# Autodesk Inventor assembly: Gantry Assembly
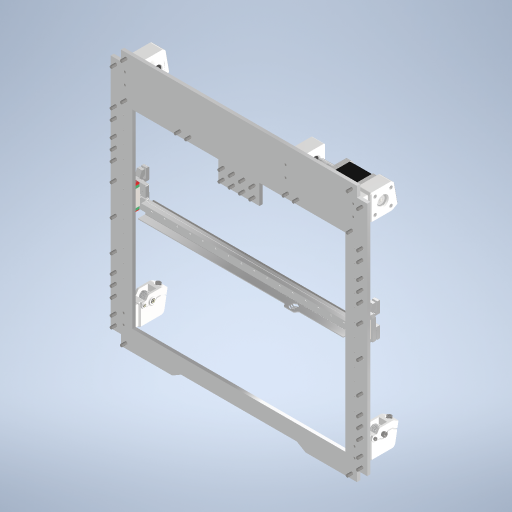
[picture p0: Inventor's stored thumbnail of the model, 512x512]
Saved by Autodesk Inventor 2024 (Build 280153000, 153)
## iProperties
Created: 2024-08-04
Part Number: Gantry Assembly
Document SubType Name: Assembly
Designer: Ishaan
Author: Ishaan
## Documents named in this file (27)
- E:\Projects\Axiom--IDEX-3D-Printer\CAD\04 - Gantry and Y-axis\Gantry Assembly.iam
- E:\Projects\Axiom--IDEX-3D-Printer\CAD\04 - Gantry and Y-axis\Printer Gantry Plate RevI.ipt
- E:\Projects\Axiom--IDEX-3D-Printer\CAD\00 - COTS Components\MGNR12 300mm Rail\MGNR12R100HM\MGNR12R100HM.ipt
- E:\Projects\Axiom--IDEX-3D-Printer\CAD\00 - COTS Components\MGN12H\MGN12H, LINEAR GUIDE BLOCK.ipt
- E:\Projects\Axiom--IDEX-3D-Printer\CAD\00 - COTS Components\MGNR12 400mm Rail\MGNR12R400HM.ipt
- E:\Projects\Axiom--IDEX-3D-Printer\CAD\04 - Gantry and Y-axis\Y-axis Motor Block.ipt
- E:\Projects\Axiom--IDEX-3D-Printer\CAD\00 - COTS Components\NEMA 17 - Y-Axis\NEMA 17 Y-axis.ipt
- E:\Projects\Axiom--IDEX-3D-Printer\CAD\00 - COTS Components\9mm 20T GT2 Timing Pulley 5mm Bore\9mm 20T GT2 Timing Pulley 5mm Bore.ipt
- E:\Projects\Axiom--IDEX-3D-Printer\CAD\04 - Gantry and Y-axis\Y-axis Bearing Pulley Block.ipt
- E:\Projects\Axiom--IDEX-3D-Printer\CAD\00 - COTS Components\608-2RS\608-2RS Bearing.ipt
- E:\Projects\Axiom--IDEX-3D-Printer\CAD\00 - COTS Components\9mm 20T GT2 Timing Pulley 8mm Bore\9mm 20T GT2 Timing Pulley 8mm Bore.ipt
- E:\Projects\Axiom--IDEX-3D-Printer\CAD\04 - Gantry and Y-axis\Y-axis Shaft Support.ipt
- E:\Projects\Axiom--IDEX-3D-Printer\CAD\00 - COTS Components\5x8 Shaft Coupler\Flexible Coupling 5mm x 8mm.ipt
- E:\Projects\Axiom--IDEX-3D-Printer\CAD\04 - Gantry and Y-axis\Y-axis Power Transfer Shaft 360mm.ipt
- E:\Projects\Axiom--IDEX-3D-Printer\CAD\04 - Gantry and Y-axis\R2 Idler Block Left.ipt
- E:\Projects\Axiom--IDEX-3D-Printer\CAD\04 - Gantry and Y-axis\R2 Idler Block Right.ipt
- E:\Projects\Axiom--IDEX-3D-Printer\CAD\00 - COTS Components\9mm 20T GT2 Idler Pulley 5mm Bore\9mm 20T GT2 Idler Pulley 5mm Bore.ipt
- E:\Projects\Axiom--IDEX-3D-Printer\CAD\04 - Gantry and Y-axis\R2 Gantry Bar.ipt
- E:\Projects\Axiom--IDEX-3D-Printer\CAD\04 - Gantry and Y-axis\Gantry Belt Clamp.ipt
- E:\Projects\Axiom--IDEX-3D-Printer\CAD\04 - Gantry and Y-axis\Gantry Stiffener.ipt
- E:\Projects\Axiom--IDEX-3D-Printer\CAD\00 - COTS Components\Hardware\Low Profile M5x16.ipt
- E:\Projects\Axiom--IDEX-3D-Printer\CAD\00 - COTS Components\Hardware\SHCSM5x16.ipt
- E:\Projects\Axiom--IDEX-3D-Printer\CAD\00 - COTS Components\Hardware\SHCSM3x8.ipt
- E:\Projects\Axiom--IDEX-3D-Printer\CAD\00 - COTS Components\Hardware\SHCSM3x25.ipt
- E:\Projects\Axiom--IDEX-3D-Printer\CAD\00 - COTS Components\Hardware\SHCSM5x25.ipt
- E:\Projects\Axiom--IDEX-3D-Printer\CAD\00 - COTS Components\Hardware\M5 LOCKNUT.ipt
- E:\Projects\Axiom--IDEX-3D-Printer\CAD\00 - COTS Components\Hardware\M3 LOCKNUT.ipt
## Components (121 placed, 26 different names)
1. Printer Gantry Plate RevI:1 — Insert:1, Insert:2, Insert:3, Insert:4, Insert:5, Insert:6, Insert:7, Insert:8, Insert:9, Insert:10, Insert:11, Insert:12, Insert:13, Insert:14, Insert:15, Insert:16, Insert:17, Insert:18, Insert:19, Insert:20, Insert:21, Insert:22, Insert:23, Insert:24, Insert:25, Flush:1, Flush:2, Insert:35, Insert:36, Insert:37, Insert:38, Insert:43, Insert:44, Insert:48, Insert:49, Insert:50, Insert:51, Insert:109, Insert:110, Insert:111, Insert:112, Insert:113, Insert:114, Insert:115, Insert:116, Insert:117, Insert:118, Insert:119, Insert:120, Insert:121, Insert:122, Insert:123, Insert:124, Insert:125, Insert:126, Insert:127, Insert:128, Insert:129, Insert:130, Insert:131, Insert:132, Insert:133, Insert:134, Insert:135, Insert:136, Insert:137, Insert:138, Insert:139, Insert:140, Insert:141, Insert:142, Insert:143, Insert:144, Insert:145, Insert:146, Insert:147, Insert:148, Insert:149, Insert:150, Insert:151, Insert:152, Insert:153, Insert:154
2. MGNR12R100HM:1 — Insert:1, Insert:14, Insert:15, Insert:16, Insert:17, Insert:18, Insert:19, Insert:20, Insert:21, Insert:22, Insert:23, Insert:24, Insert:25, Mate:2, Flush:3, Flush:4, Insert:165, Insert:166, Insert:167, Insert:168, Insert:169, Insert:170, Insert:171, Insert:172, Insert:173, Insert:174, Insert:175, Insert:176
3. MGNR12R100HM:2 — Insert:2, Insert:3, Insert:4, Insert:5, Insert:6, Insert:7, Insert:8, Insert:9, Insert:10, Insert:11, Insert:12, Insert:13, Mate:4, Insert:177, Insert:178, Insert:179, Insert:180, Insert:181, Insert:182, Insert:183, Insert:184, Insert:185, Insert:186, Insert:187, Insert:188
4. MGN12H, LINEAR GUIDE BLOCK:1 — Mate:2, Flush:1, Insert:64, Insert:65, Insert:66, Insert:67, Flush:3, Flush:4
5. MGN12H, LINEAR GUIDE BLOCK:2 — Mate:4, Flush:2, Insert:68, Insert:69, Insert:70, Insert:71
6. MGNR12R400HM:1 — Insert:72, Insert:73, Insert:74, Insert:75, Insert:76, Insert:77, Insert:78, Insert:79, Insert:80, Insert:81, Insert:82, Insert:83, Insert:84, Insert:85, Insert:86, Insert:87, Insert:88
7. Y-axis Motor Block:1 — Insert:32, Insert:33, Insert:35, Insert:36, Insert:163, Insert:164, Insert:189, Insert:190, Insert:191, Insert:192
8. NEMA 17 Y-axis:1 — Insert:32, Insert:33, Insert:34, Insert:46
9. 9mm 20T GT2 Timing Pulley 5mm Bore:1 — Insert:34
10. Y-axis Bearing Pulley Block:1 — Insert:37, Insert:38, Insert:39, Insert:40, Insert:159, Insert:160
11. 608-2RS Bearing:1 — Insert:40, Insert:41
12. 608-2RS Bearing:2 — Insert:39, Insert:42, Insert:47
13. 9mm 20T GT2 Timing Pulley 8mm Bore:1 — Insert:41, Insert:42
14. Y-axis Shaft Support:1 — Insert:43, Insert:44, Insert:45, Insert:161, Insert:162
15. 608-2RS Bearing:3 — Insert:45, Mate:5
16. Flexible Coupling 5mm x 8mm:1 — Insert:46
17. Y-axis Power Transfer Shaft 360mm:1 — Insert:47, Mate:5
18. R2 Gantry Bar:1 — Insert:64, Insert:65, Insert:66, Insert:67, Insert:68, Insert:69, Insert:70, Insert:71, Insert:72, Insert:73, Insert:74, Insert:75, Insert:76, Insert:77, Insert:78, Insert:79, Insert:80, Insert:81, Insert:82, Insert:83, Insert:84, Insert:85, Insert:86, Insert:87, Insert:88, Insert:89, Insert:90, Insert:91, Insert:92, Insert:93, Insert:94, Insert:95, Insert:96, Insert:97, Insert:98, Insert:99, Insert:100, Insert:101, Insert:102, Insert:103, Insert:104, Insert:105, Insert:106, Insert:107, Insert:108
19. Gantry Belt Clamp:1 — Insert:91, Insert:92
20. Gantry Belt Clamp:2 — Insert:89, Insert:90
21. Gantry Stiffener:1 — Insert:93, Insert:94, Insert:95, Insert:96, Insert:97, Insert:98, Insert:99, Insert:100, Insert:101, Insert:102, Insert:103, Insert:104, Insert:105, Insert:106, Insert:107, Insert:108
22. Low Profile M5x16:1 — Insert:109
23. Low Profile M5x16:2 — Insert:110
24. Low Profile M5x16:3 — Insert:111
25. Low Profile M5x16:4 — Insert:112
26. Low Profile M5x16:5 — Insert:113
27. Low Profile M5x16:6 — Insert:114
28. Low Profile M5x16:7 — Insert:116
29. Low Profile M5x16:8 — Insert:118
30. Low Profile M5x16:9 — Insert:115
31. Low Profile M5x16:10 — Insert:117
32. Low Profile M5x16:11 — Insert:119
33. Low Profile M5x16:12 — Insert:120
34. Low Profile M5x16:13 — Insert:121
35. Low Profile M5x16:14 — Insert:122
36. Low Profile M5x16:15 — Insert:123
37. Low Profile M5x16:16 — Insert:124
38. Low Profile M5x16:17 — Insert:125
39. Low Profile M5x16:18 — Insert:126
40. Low Profile M5x16:19 — Insert:127
41. Low Profile M5x16:20 — Insert:128
42. Low Profile M5x16:21 — Insert:129
43. Low Profile M5x16:22 — Insert:130
44. Low Profile M5x16:23 — Insert:131
45. Low Profile M5x16:24 — Insert:133
46. Low Profile M5x16:25 — Insert:135
47. Low Profile M5x16:26 — Insert:132
48. Low Profile M5x16:27 — Insert:134
49. Low Profile M5x16:28 — Insert:136
50. Low Profile M5x16:29 — Insert:137
51. Low Profile M5x16:30 — Insert:138
52. Low Profile M5x16:31 — Insert:139
53. Low Profile M5x16:32 — Insert:140
54. Low Profile M5x16:33 — Insert:141
55. Low Profile M5x16:34 — Insert:142
56. Low Profile M5x16:35 — Insert:143
57. Low Profile M5x16:36 — Insert:144
58. Low Profile M5x16:37 — Insert:145
59. Low Profile M5x16:38 — Insert:146
60. Low Profile M5x16:39 — Insert:147
61. Low Profile M5x16:40 — Insert:148
62. Low Profile M5x16:41 — Insert:149
63. Low Profile M5x16:42 — Insert:150
64. Low Profile M5x16:43 — Insert:151
65. Low Profile M5x16:44 — Insert:152
66. Low Profile M5x16:45 — Insert:153
67. Low Profile M5x16:46 — Insert:154
68. SHCSM5x16:1 — Insert:155
69. SHCSM5x16:2 — Insert:156
70. SHCSM5x16:3 — Insert:158
71. SHCSM5x16:4 — Insert:160
72. SHCSM5x16:5 — Insert:163
73. SHCSM5x16:6 — Insert:164
74. SHCSM5x16:7 — Insert:162
75. SHCSM5x16:8 — Insert:161
76. SHCSM5x16:9 — Insert:159
77. SHCSM5x16:10 — Insert:157
78. SHCSM3x8:1 — Insert:165
79. SHCSM3x8:2 — Insert:166
80. SHCSM3x8:3 — Insert:167
81. SHCSM3x8:4 — Insert:168
82. SHCSM3x8:5 — Insert:169
83. SHCSM3x8:6 — Insert:170
84. SHCSM3x8:7 — Insert:171
85. SHCSM3x8:8 — Insert:172
86. SHCSM3x8:9 — Insert:173
87. SHCSM3x8:10 — Insert:174
88. SHCSM3x8:11 — Insert:175
89. SHCSM3x8:12 — Insert:176
90. SHCSM3x8:13 — Insert:177
91. SHCSM3x8:14 — Insert:178
92. SHCSM3x8:15 — Insert:179
93. SHCSM3x8:16 — Insert:180
94. SHCSM3x8:17 — Insert:181
95. SHCSM3x8:18 — Insert:182
96. SHCSM3x8:19 — Insert:183
97. SHCSM3x8:20 — Insert:184
98. SHCSM3x8:21 — Insert:185
99. SHCSM3x8:22 — Insert:186
100. SHCSM3x8:23 — Insert:187
101. SHCSM3x8:24 — Insert:188
102. SHCSM3x25:1 — Insert:189
103. SHCSM3x25:2 — Insert:190
104. SHCSM3x25:3 — Insert:192
105. SHCSM3x25:4 — Insert:191
106. SHCSM3x25:5 — Insert:193
107. SHCSM3x25:6 — Insert:194
108. SHCSM5x25:1 — Insert:195
109. SHCSM5x25:2 — Insert:196
110. SHCSM5x25:3 — Mate:7, Mate:9
111. SHCSM5x25:4 — Mate:6, Mate:8
112. M5 LOCKNUT:1 — Insert:197, Angle:3
113. M5 LOCKNUT:2 — Insert:198, Angle:4
114. M5 LOCKNUT:3 — Insert:199, Angle:2
115. M5 LOCKNUT:4 — Insert:200, Angle:1
116. M3 LOCKNUT:1 — Insert:201, Angle:6
117. M3 LOCKNUT:2 — Insert:202, Angle:5
118. R2 Idler Block Left:1 — Insert:48, Insert:49, Insert:54, Insert:55, Insert:157, Insert:158, Insert:193, Insert:195, Mate:6, Mate:8, Insert:197, Insert:198, Angle:3, Angle:4, Insert:202, Angle:5
119. R2 Idler Block Right:1 — Insert:50, Insert:51, Insert:52, Insert:53, Insert:155, Insert:156, Insert:194, Insert:196, Mate:7, Mate:9, Insert:199, Insert:200, Angle:1, Angle:2, Insert:201, Angle:6
120. 9mm 20T GT2 Idler Pulley 5mm Bore:1 — Insert:52, Insert:53
121. 9mm 20T GT2 Idler Pulley 5mm Bore:2 — Insert:54, Insert:55
## Relationships (205: Insert 188, Mate 7, Angle 6, Flush 4)
- Insert:1: Printer Gantry Plate RevI:1 ↔ MGNR12R100HM:1
- Insert:2: Printer Gantry Plate RevI:1 ↔ MGNR12R100HM:2
- Insert:3: Printer Gantry Plate RevI:1 ↔ MGNR12R100HM:2
- Insert:4: Printer Gantry Plate RevI:1 ↔ MGNR12R100HM:2
- Insert:5: Printer Gantry Plate RevI:1 ↔ MGNR12R100HM:2
- Insert:6: Printer Gantry Plate RevI:1 ↔ MGNR12R100HM:2
- Insert:7: Printer Gantry Plate RevI:1 ↔ MGNR12R100HM:2
- Insert:8: Printer Gantry Plate RevI:1 ↔ MGNR12R100HM:2
- Insert:9: Printer Gantry Plate RevI:1 ↔ MGNR12R100HM:2
- Insert:10: Printer Gantry Plate RevI:1 ↔ MGNR12R100HM:2
- Insert:11: Printer Gantry Plate RevI:1 ↔ MGNR12R100HM:2
- Insert:12: Printer Gantry Plate RevI:1 ↔ MGNR12R100HM:2
- Insert:13: Printer Gantry Plate RevI:1 ↔ MGNR12R100HM:2
- Insert:14: Printer Gantry Plate RevI:1 ↔ MGNR12R100HM:1
- Insert:15: Printer Gantry Plate RevI:1 ↔ MGNR12R100HM:1
- Insert:16: Printer Gantry Plate RevI:1 ↔ MGNR12R100HM:1
- Insert:17: Printer Gantry Plate RevI:1 ↔ MGNR12R100HM:1
- Insert:18: Printer Gantry Plate RevI:1 ↔ MGNR12R100HM:1
- Insert:19: Printer Gantry Plate RevI:1 ↔ MGNR12R100HM:1
- Insert:20: Printer Gantry Plate RevI:1 ↔ MGNR12R100HM:1
- Insert:21: Printer Gantry Plate RevI:1 ↔ MGNR12R100HM:1
- Insert:22: Printer Gantry Plate RevI:1 ↔ MGNR12R100HM:1
- Insert:23: Printer Gantry Plate RevI:1 ↔ MGNR12R100HM:1
- Insert:24: Printer Gantry Plate RevI:1 ↔ MGNR12R100HM:1
- Insert:25: Printer Gantry Plate RevI:1 ↔ MGNR12R100HM:1
- Mate:2: MGNR12R100HM:1 ↔ MGN12H, LINEAR GUIDE BLOCK:1
- Mate:4: MGNR12R100HM:2 ↔ MGN12H, LINEAR GUIDE BLOCK:2
- Flush:1 (13 mm): Printer Gantry Plate RevI:1 ↔ MGN12H, LINEAR GUIDE BLOCK:1
- Flush:2 (13 mm): Printer Gantry Plate RevI:1 ↔ MGN12H, LINEAR GUIDE BLOCK:2
- Insert:32: Y-axis Motor Block:1 ↔ NEMA 17 Y-axis:1
- Insert:33: Y-axis Motor Block:1 ↔ NEMA 17 Y-axis:1
- Insert:34: NEMA 17 Y-axis:1 ↔ 9mm 20T GT2 Timing Pulley 5mm Bore:1
- Insert:35: Printer Gantry Plate RevI:1 ↔ Y-axis Motor Block:1
- Insert:36: Printer Gantry Plate RevI:1 ↔ Y-axis Motor Block:1
- Insert:37: Printer Gantry Plate RevI:1 ↔ Y-axis Bearing Pulley Block:1
- Insert:38: Printer Gantry Plate RevI:1 ↔ Y-axis Bearing Pulley Block:1
- Insert:39: Y-axis Bearing Pulley Block:1 ↔ 608-2RS Bearing:2
- Insert:40: Y-axis Bearing Pulley Block:1 ↔ 608-2RS Bearing:1
- Insert:41 (0.5 mm): 608-2RS Bearing:1 ↔ 9mm 20T GT2 Timing Pulley 8mm Bore:1
- Insert:42 (0.5 mm): 608-2RS Bearing:2 ↔ 9mm 20T GT2 Timing Pulley 8mm Bore:1
- Insert:43: Printer Gantry Plate RevI:1 ↔ Y-axis Shaft Support:1
- Insert:44: Printer Gantry Plate RevI:1 ↔ Y-axis Shaft Support:1
- Insert:45: Y-axis Shaft Support:1 ↔ 608-2RS Bearing:3
- Insert:46: NEMA 17 Y-axis:1 ↔ Flexible Coupling 5mm x 8mm:1
- Insert:47 (-1 mm): 608-2RS Bearing:2 ↔ Y-axis Power Transfer Shaft 360mm:1
- Mate:5: 608-2RS Bearing:3 ↔ Y-axis Power Transfer Shaft 360mm:1
- Insert:48: Printer Gantry Plate RevI:1 ↔ R2 Idler Block Left:1
- Insert:49: Printer Gantry Plate RevI:1 ↔ R2 Idler Block Left:1
- Insert:50: Printer Gantry Plate RevI:1 ↔ R2 Idler Block Right:1
- Insert:51: Printer Gantry Plate RevI:1 ↔ R2 Idler Block Right:1
- Insert:52 (0.5 mm): R2 Idler Block Right:1 ↔ 9mm 20T GT2 Idler Pulley 5mm Bore:1
- Insert:53 (0.5 mm): R2 Idler Block Right:1 ↔ 9mm 20T GT2 Idler Pulley 5mm Bore:1
- Insert:54 (0.5 mm): R2 Idler Block Left:1 ↔ 9mm 20T GT2 Idler Pulley 5mm Bore:2
- Insert:55 (0.5 mm): R2 Idler Block Left:1 ↔ 9mm 20T GT2 Idler Pulley 5mm Bore:2
- Insert:64: MGN12H, LINEAR GUIDE BLOCK:1 ↔ R2 Gantry Bar:1
- Insert:65: MGN12H, LINEAR GUIDE BLOCK:1 ↔ R2 Gantry Bar:1
- Insert:66: MGN12H, LINEAR GUIDE BLOCK:1 ↔ R2 Gantry Bar:1
- Insert:67: MGN12H, LINEAR GUIDE BLOCK:1 ↔ R2 Gantry Bar:1
- Insert:68: MGN12H, LINEAR GUIDE BLOCK:2 ↔ R2 Gantry Bar:1
- Insert:69: MGN12H, LINEAR GUIDE BLOCK:2 ↔ R2 Gantry Bar:1
- Insert:70: MGN12H, LINEAR GUIDE BLOCK:2 ↔ R2 Gantry Bar:1
- Insert:71: MGN12H, LINEAR GUIDE BLOCK:2 ↔ R2 Gantry Bar:1
- Insert:72: MGNR12R400HM:1 ↔ R2 Gantry Bar:1
- Insert:73: MGNR12R400HM:1 ↔ R2 Gantry Bar:1
- Insert:74: MGNR12R400HM:1 ↔ R2 Gantry Bar:1
- Insert:75: MGNR12R400HM:1 ↔ R2 Gantry Bar:1
- Insert:76: MGNR12R400HM:1 ↔ R2 Gantry Bar:1
- Insert:77: MGNR12R400HM:1 ↔ R2 Gantry Bar:1
- Insert:78: MGNR12R400HM:1 ↔ R2 Gantry Bar:1
- Insert:79: MGNR12R400HM:1 ↔ R2 Gantry Bar:1
- Insert:80: MGNR12R400HM:1 ↔ R2 Gantry Bar:1
- Insert:81: MGNR12R400HM:1 ↔ R2 Gantry Bar:1
- Insert:82: MGNR12R400HM:1 ↔ R2 Gantry Bar:1
- Insert:83: MGNR12R400HM:1 ↔ R2 Gantry Bar:1
- Insert:84: MGNR12R400HM:1 ↔ R2 Gantry Bar:1
- Insert:85: MGNR12R400HM:1 ↔ R2 Gantry Bar:1
- Insert:86: MGNR12R400HM:1 ↔ R2 Gantry Bar:1
- Insert:87: MGNR12R400HM:1 ↔ R2 Gantry Bar:1
- Insert:88: MGNR12R400HM:1 ↔ R2 Gantry Bar:1
- Flush:3: MGNR12R100HM:1 ↔ MGN12H, LINEAR GUIDE BLOCK:1
- Flush:4: MGNR12R100HM:1 ↔ MGN12H, LINEAR GUIDE BLOCK:1
- Insert:89 (0.1 mm): R2 Gantry Bar:1 ↔ Gantry Belt Clamp:2
- Insert:90 (0.1 mm): R2 Gantry Bar:1 ↔ Gantry Belt Clamp:2
- Insert:91 (0.1 mm): R2 Gantry Bar:1 ↔ Gantry Belt Clamp:1
- Insert:92 (0.1 mm): R2 Gantry Bar:1 ↔ Gantry Belt Clamp:1
- Insert:93: R2 Gantry Bar:1 ↔ Gantry Stiffener:1
- Insert:94: R2 Gantry Bar:1 ↔ Gantry Stiffener:1
- Insert:95: R2 Gantry Bar:1 ↔ Gantry Stiffener:1
- Insert:96: R2 Gantry Bar:1 ↔ Gantry Stiffener:1
- Insert:97: R2 Gantry Bar:1 ↔ Gantry Stiffener:1
- Insert:98: R2 Gantry Bar:1 ↔ Gantry Stiffener:1
- Insert:99: R2 Gantry Bar:1 ↔ Gantry Stiffener:1
- Insert:100: R2 Gantry Bar:1 ↔ Gantry Stiffener:1
- Insert:101: R2 Gantry Bar:1 ↔ Gantry Stiffener:1
- Insert:102: R2 Gantry Bar:1 ↔ Gantry Stiffener:1
- Insert:103: R2 Gantry Bar:1 ↔ Gantry Stiffener:1
- Insert:104: R2 Gantry Bar:1 ↔ Gantry Stiffener:1
- Insert:105: R2 Gantry Bar:1 ↔ Gantry Stiffener:1
- Insert:106: R2 Gantry Bar:1 ↔ Gantry Stiffener:1
- Insert:107: R2 Gantry Bar:1 ↔ Gantry Stiffener:1
- Insert:108: R2 Gantry Bar:1 ↔ Gantry Stiffener:1
- Insert:109: Printer Gantry Plate RevI:1 ↔ Low Profile M5x16:1
- Insert:110: Printer Gantry Plate RevI:1 ↔ Low Profile M5x16:2
- Insert:111: Printer Gantry Plate RevI:1 ↔ Low Profile M5x16:3
- Insert:112: Printer Gantry Plate RevI:1 ↔ Low Profile M5x16:4
- Insert:113: Printer Gantry Plate RevI:1 ↔ Low Profile M5x16:5
- Insert:114: Printer Gantry Plate RevI:1 ↔ Low Profile M5x16:6
- Insert:115: Printer Gantry Plate RevI:1 ↔ Low Profile M5x16:9
- Insert:116: Printer Gantry Plate RevI:1 ↔ Low Profile M5x16:7
- Insert:117: Printer Gantry Plate RevI:1 ↔ Low Profile M5x16:10
- Insert:118: Printer Gantry Plate RevI:1 ↔ Low Profile M5x16:8
- Insert:119: Printer Gantry Plate RevI:1 ↔ Low Profile M5x16:11
- Insert:120: Printer Gantry Plate RevI:1 ↔ Low Profile M5x16:12
- Insert:121: Printer Gantry Plate RevI:1 ↔ Low Profile M5x16:13
- Insert:122: Printer Gantry Plate RevI:1 ↔ Low Profile M5x16:14
- Insert:123: Printer Gantry Plate RevI:1 ↔ Low Profile M5x16:15
- Insert:124: Printer Gantry Plate RevI:1 ↔ Low Profile M5x16:16
- Insert:125: Printer Gantry Plate RevI:1 ↔ Low Profile M5x16:17
- Insert:126: Printer Gantry Plate RevI:1 ↔ Low Profile M5x16:18
- Insert:127: Printer Gantry Plate RevI:1 ↔ Low Profile M5x16:19
- Insert:128: Printer Gantry Plate RevI:1 ↔ Low Profile M5x16:20
- Insert:129: Printer Gantry Plate RevI:1 ↔ Low Profile M5x16:21
- Insert:130: Printer Gantry Plate RevI:1 ↔ Low Profile M5x16:22
- Insert:131: Printer Gantry Plate RevI:1 ↔ Low Profile M5x16:23
- Insert:132: Printer Gantry Plate RevI:1 ↔ Low Profile M5x16:26
- Insert:133: Printer Gantry Plate RevI:1 ↔ Low Profile M5x16:24
- Insert:134: Printer Gantry Plate RevI:1 ↔ Low Profile M5x16:27
- Insert:135: Printer Gantry Plate RevI:1 ↔ Low Profile M5x16:25
- Insert:136: Printer Gantry Plate RevI:1 ↔ Low Profile M5x16:28
- Insert:137: Printer Gantry Plate RevI:1 ↔ Low Profile M5x16:29
- Insert:138: Printer Gantry Plate RevI:1 ↔ Low Profile M5x16:30
- Insert:139: Printer Gantry Plate RevI:1 ↔ Low Profile M5x16:31
- Insert:140: Printer Gantry Plate RevI:1 ↔ Low Profile M5x16:32
- Insert:141: Printer Gantry Plate RevI:1 ↔ Low Profile M5x16:33
- Insert:142: Printer Gantry Plate RevI:1 ↔ Low Profile M5x16:34
- Insert:143: Printer Gantry Plate RevI:1 ↔ Low Profile M5x16:35
- Insert:144: Printer Gantry Plate RevI:1 ↔ Low Profile M5x16:36
- Insert:145: Printer Gantry Plate RevI:1 ↔ Low Profile M5x16:37
- Insert:146: Printer Gantry Plate RevI:1 ↔ Low Profile M5x16:38
- Insert:147: Printer Gantry Plate RevI:1 ↔ Low Profile M5x16:39
- Insert:148: Printer Gantry Plate RevI:1 ↔ Low Profile M5x16:40
- Insert:149: Printer Gantry Plate RevI:1 ↔ Low Profile M5x16:41
- Insert:150: Printer Gantry Plate RevI:1 ↔ Low Profile M5x16:42
- Insert:151: Printer Gantry Plate RevI:1 ↔ Low Profile M5x16:43
- Insert:152: Printer Gantry Plate RevI:1 ↔ Low Profile M5x16:44
- Insert:153: Printer Gantry Plate RevI:1 ↔ Low Profile M5x16:45
- Insert:154: Printer Gantry Plate RevI:1 ↔ Low Profile M5x16:46
- Insert:155: SHCSM5x16:1 ↔ R2 Idler Block Right:1
- Insert:156: SHCSM5x16:2 ↔ R2 Idler Block Right:1
- Insert:157: SHCSM5x16:10 ↔ R2 Idler Block Left:1
- Insert:158: SHCSM5x16:3 ↔ R2 Idler Block Left:1
- Insert:159: Y-axis Bearing Pulley Block:1 ↔ SHCSM5x16:9
- Insert:160: Y-axis Bearing Pulley Block:1 ↔ SHCSM5x16:4
- Insert:161: Y-axis Shaft Support:1 ↔ SHCSM5x16:8
- Insert:162: Y-axis Shaft Support:1 ↔ SHCSM5x16:7
- Insert:163: Y-axis Motor Block:1 ↔ SHCSM5x16:5
- Insert:164: Y-axis Motor Block:1 ↔ SHCSM5x16:6
- Insert:165: MGNR12R100HM:1 ↔ SHCSM3x8:1
- Insert:166: MGNR12R100HM:1 ↔ SHCSM3x8:2
- Insert:167: MGNR12R100HM:1 ↔ SHCSM3x8:3
- Insert:168: MGNR12R100HM:1 ↔ SHCSM3x8:4
- Insert:169: MGNR12R100HM:1 ↔ SHCSM3x8:5
- Insert:170: MGNR12R100HM:1 ↔ SHCSM3x8:6
- Insert:171: MGNR12R100HM:1 ↔ SHCSM3x8:7
- Insert:172: MGNR12R100HM:1 ↔ SHCSM3x8:8
- Insert:173: MGNR12R100HM:1 ↔ SHCSM3x8:9
- Insert:174: MGNR12R100HM:1 ↔ SHCSM3x8:10
- Insert:175: MGNR12R100HM:1 ↔ SHCSM3x8:11
- Insert:176: MGNR12R100HM:1 ↔ SHCSM3x8:12
- Insert:177: MGNR12R100HM:2 ↔ SHCSM3x8:13
- Insert:178: MGNR12R100HM:2 ↔ SHCSM3x8:14
- Insert:179: MGNR12R100HM:2 ↔ SHCSM3x8:15
- Insert:180: MGNR12R100HM:2 ↔ SHCSM3x8:16
- Insert:181: MGNR12R100HM:2 ↔ SHCSM3x8:17
- Insert:182: MGNR12R100HM:2 ↔ SHCSM3x8:18
- Insert:183: MGNR12R100HM:2 ↔ SHCSM3x8:19
- Insert:184: MGNR12R100HM:2 ↔ SHCSM3x8:20
- Insert:185: MGNR12R100HM:2 ↔ SHCSM3x8:21
- Insert:186: MGNR12R100HM:2 ↔ SHCSM3x8:22
- Insert:187: MGNR12R100HM:2 ↔ SHCSM3x8:23
- Insert:188: MGNR12R100HM:2 ↔ SHCSM3x8:24
- Insert:189: Y-axis Motor Block:1 ↔ SHCSM3x25:1
- Insert:190: Y-axis Motor Block:1 ↔ SHCSM3x25:2
- Insert:191: Y-axis Motor Block:1 ↔ SHCSM3x25:4
- Insert:192: Y-axis Motor Block:1 ↔ SHCSM3x25:3
- Insert:193: SHCSM3x25:5 ↔ R2 Idler Block Left:1
- Insert:194: SHCSM3x25:6 ↔ R2 Idler Block Right:1
- Insert:195: SHCSM5x25:1 ↔ R2 Idler Block Left:1
- Insert:196: SHCSM5x25:2 ↔ R2 Idler Block Right:1
- Mate:6: SHCSM5x25:4 ↔ R2 Idler Block Left:1
- Mate:7: SHCSM5x25:3 ↔ R2 Idler Block Right:1
- Mate:8: SHCSM5x25:4 ↔ R2 Idler Block Left:1
- Mate:9: SHCSM5x25:3 ↔ R2 Idler Block Right:1
- Insert:197: M5 LOCKNUT:1 ↔ R2 Idler Block Left:1
- Insert:198: M5 LOCKNUT:2 ↔ R2 Idler Block Left:1
- Insert:199: M5 LOCKNUT:3 ↔ R2 Idler Block Right:1
- Insert:200: M5 LOCKNUT:4 ↔ R2 Idler Block Right:1
- Angle:1 (0 deg): M5 LOCKNUT:4 ↔ R2 Idler Block Right:1
- Angle:2 (0 deg): M5 LOCKNUT:3 ↔ R2 Idler Block Right:1
- Angle:3 (0 deg): M5 LOCKNUT:1 ↔ R2 Idler Block Left:1
- Angle:4 (0 deg): M5 LOCKNUT:2 ↔ R2 Idler Block Left:1
- Insert:201: M3 LOCKNUT:1 ↔ R2 Idler Block Right:1
- Insert:202: M3 LOCKNUT:2 ↔ R2 Idler Block Left:1
- Angle:5 (0 deg): M3 LOCKNUT:2 ↔ R2 Idler Block Left:1
- Angle:6 (0 deg): M3 LOCKNUT:1 ↔ R2 Idler Block Right:1
